# Autodesk Inventor assembly: CanSat
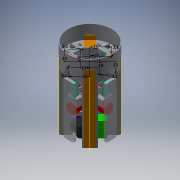
[picture p0: Inventor's stored thumbnail of the model, 180x180]
Saved by Autodesk Inventor 2018.2 (Build 222227000, 227)
## iProperties
Created: 2018-05-01
Part Number: CanSat
Document SubType Name: Assembly
Designer: suchanek
Author: suchanek
## Documents named in this file (25)
- C:\Users\Kuba\Documents\GitHub\CanSatGOSA\CanSat2.0\Schematics\Model\CanSat.iam
- C:\Users\Kuba\Documents\GitHub\CanSatGOSA\CanSat2.0\Schematics\Model\Hull_middle.ipt
- C:\Users\Kuba\Documents\GitHub\CanSatGOSA\CanSat2.0\Schematics\Model\Hull_batt_pillar.ipt
- C:\Users\Kuba\Documents\GitHub\CanSatGOSA\CanSat2.0\Schematics\Model\Circuit.ipt
- C:\Users\Kuba\Documents\GitHub\CanSatGOSA\CanSat2.0\Schematics\Model\Motor_drivers.ipt
- C:\Users\Kuba\Documents\GitHub\CanSatGOSA\CanSat2.0\Schematics\Model\Hull_main.ipt
- C:\Users\Kuba\Documents\GitHub\CanSatGOSA\CanSat2.0\Schematics\Model\Circuit_center.ipt
- C:\Users\Kuba\Documents\GitHub\CanSatGOSA\CanSat2.0\Schematics\Model\Arm.ipt
- C:\Users\Kuba\Documents\GitHub\CanSatGOSA\CanSat2.0\Schematics\Model\Motor_holder.ipt
- C:\Users\Kuba\Documents\GitHub\CanSatGOSA\CanSat2.0\Schematics\Model\Motor.ipt
- C:\Users\Kuba\Documents\GitHub\CanSatGOSA\CanSat2.0\Schematics\Model\Rotor.ipt
- C:\Users\Kuba\Documents\GitHub\CanSatGOSA\CanSat2.0\Schematics\Model\Flight_controler.ipt
- C:\Users\Kuba\Documents\GitHub\CanSatGOSA\CanSat2.0\Schematics\Model\SIM808.ipt
- C:\Users\Kuba\Documents\GitHub\CanSatGOSA\CanSat2.0\Schematics\Model\Batt_pillar.ipt
- C:\Users\Kuba\Documents\GitHub\CanSatGOSA\CanSat2.0\Schematics\Model\Servo.ipt
- C:\Users\Kuba\Documents\GitHub\CanSatGOSA\CanSat2.0\Schematics\Model\Servo_bit.ipt
- C:\Users\Kuba\Documents\GitHub\CanSatGOSA\CanSat2.0\Schematics\Model\Spring.ipt
- C:\Users\Kuba\Documents\GitHub\CanSatGOSA\CanSat2.0\Schematics\Model\Scraper.ipt
- C:\Users\Kuba\Documents\GitHub\CanSatGOSA\CanSat2.0\Schematics\Model\Camera.ipt
- C:\Users\Kuba\Documents\GitHub\CanSatGOSA\CanSat2.0\Schematics\Model\Cam_SD_base.ipt
- C:\Users\Kuba\Documents\GitHub\CanSatGOSA\CanSat2.0\Schematics\Model\Cam_SD_chip.ipt
- C:\Users\Kuba\Documents\GitHub\CanSatGOSA\CanSat2.0\Schematics\Model\Hull_batt_pillar1.ipt
- C:\Users\Kuba\Documents\GitHub\CanSatGOSA\CanSat2.0\Schematics\Model\Hull_batt_pillar3.ipt
- C:\Users\Kuba\Documents\GitHub\CanSatGOSA\CanSat2.0\Schematics\Model\Hull_batt_pillar2.ipt
- C:\Users\Kuba\Documents\GitHub\CanSatGOSA\CanSat2.0\Schematics\Model\Hull_batt_pillar4.ipt
## Components (42 placed, 24 different names)
1. Hull_middle:1 — Rotational:2, Angle:2, Rotational:3, Flush:2, Mate:9
2. Circuit:1 — Rotational:2, Angle:2, Angle:3
3. Motor_drivers:1 — Flush:1, Angle:4, Cylindrical:1, Mate:1
4. Hull_main:1 — Rotational:1, Angle:1, Rotational:3, Angle:3, Flush:1, Angle:4, Cylindrical:1, Rotational:4, Mate:3, Mate:6, Tangent:1, Rotační:8, Rotační:9, Rotační:10, Rotační:11, Rotační:12, Rotační:13, Rotační:14
5. Circuit_center:1 — Flush:2, Mate:9, Tangent:1
6. Flight_controler:1 — Mate:1, Mate:2, Flush:4, Symmetry:1
7. SIM808:1 — Mate:2, Flush:4, Symmetry:1, Mate:7
8. Servo:1 — Rotational:6, Mate:8, Flush:6, Flush:11
9. Servo_bit:1 — Rotational:6, Rigid:3, Angle:11
10. Spring:1 — Rigid:3, Rotational:7
11. Scraper:1 — Rotational:7, Angle:11
12. Camera:1 — Flush:7, Flush:11
13. Cam_SD_base:1 — Flush:8, Angle:12, Flush:10, Angle:13
14. Cam_SD_chip:1 — Flush:10, Angle:13
15. Hull_batt_pillar1:1 — Rotační:8
16. Hull_batt_pillar3:1 — Rotační:9, Rotační:10
17. Hull_batt_pillar2:1 — Rotační:11, Rotační:12
18. Hull_batt_pillar4:1 — Rotační:13, Rotační:14
19. Batt_pillar:1 — Cylindrical:2, Mate:6, Angle:8
20. Hull_batt_pillar:1 — Rotational:1, Angle:1, Cylindrical:2, Angle:8, Angle:10
21. Batt_pillar:2 — Flush:8, Angle:12
22. Hull_batt_pillar:2
23. Batt_pillar:3
24. Hull_batt_pillar:3 — Mate:7
25. Batt_pillar:4
26. Hull_batt_pillar:4 — Angle:9, Mate:8, Flush:6, Flush:7
27. Arm:1 — Rotational:4, Rigid:1
28. Motor_holder:1 — Rigid:1, Rigid:2
29. Motor:1 — Rigid:2, Rotational:5
30. Rotor:1 — Rotational:5
31. Arm:2
32. Motor_holder:2
33. Motor:2
34. Rotor:2
35. Arm:3
36. Motor_holder:3
37. Motor:3
38. Rotor:3
39. Arm:4
40. Motor_holder:4
41. Motor:4
42. Rotor:4
## Component patterns: (4 elements, first: Batt_pillar:1 + Hull_batt_pillar:1), (4 elements, first: Arm:1 + Motor_holder:1 + Motor:1 + Rotor:1)
## Relationships (48: RevoluteJoint 14, Angle 10, Mate 9, Flush 8, WeldJoint 3, CylindricalJoint 2, Symmetry 1, Tangent 1)
- Rotational:1 [RevoluteJoint]: Hull_main:1 ↔ Hull_batt_pillar:1
- Angle:1 (0 deg): Hull_main:1 ↔ Hull_batt_pillar:1
- Rotational:2 [RevoluteJoint]: Hull_middle:1 ↔ Circuit:1
- Angle:2 (0 deg): Hull_middle:1 ↔ Circuit:1
- Rotational:3 [RevoluteJoint]: Hull_middle:1 ↔ Hull_main:1
- Angle:3 (0 deg): Circuit:1 ↔ Hull_main:1
- Flush:1 (12 mm): Motor_drivers:1 ↔ Hull_main:1
- Angle:4 (0 deg): Motor_drivers:1 ↔ Hull_main:1
- Cylindrical:1: Motor_drivers:1 ↔ Hull_main:1
- Flush:2 (3 mm): Hull_middle:1 ↔ Circuit_center:1
- Rotational:4 [RevoluteJoint] (-0.15 mm): Hull_main:1 ↔ Arm:1
- Rigid:1 [WeldJoint]: Arm:1 ↔ Motor_holder:1
- Rigid:2 [WeldJoint]: Motor_holder:1 ↔ Motor:1
- Rotational:5 [RevoluteJoint]: Motor:1 ↔ Rotor:1
- Mate:1 (5 mm): Motor_drivers:1 ↔ Flight_controler:1
- Mate:2 (2 mm): Flight_controler:1 ↔ SIM808:1
- Mate:3: Hull_main:1
- Mate:4
- Mate:5
- Flush:4 (-0.5 mm): Flight_controler:1 ↔ SIM808:1
- Cylindrical:2: Batt_pillar:1 ↔ Hull_batt_pillar:1
- Mate:6: Hull_main:1 ↔ Batt_pillar:1
- Angle:8 (0 deg): Batt_pillar:1 ↔ Hull_batt_pillar:1
- Angle:9 (0 deg): Hull_batt_pillar:4
- Angle:10 (0 deg): Hull_batt_pillar:1
- Symmetry:1: Flight_controler:1 ↔ SIM808:1
- Mate:7: SIM808:1 ↔ Hull_batt_pillar:3
- Rotational:6 [RevoluteJoint]: Servo:1 ↔ Servo_bit:1
- Rigid:3 [WeldJoint]: Servo_bit:1 ↔ Spring:1
- Rotational:7 [RevoluteJoint]: Spring:1 ↔ Scraper:1
- Angle:11 (0 deg): Servo_bit:1 ↔ Scraper:1
- Mate:8: Servo:1 ↔ Hull_batt_pillar:4
- Flush:6: Servo:1 ↔ Hull_batt_pillar:4
- Flush:7: Camera:1 ↔ Hull_batt_pillar:4
- Flush:8: Cam_SD_base:1 ↔ Batt_pillar:2
- Angle:12 (0 deg): Cam_SD_base:1 ↔ Batt_pillar:2
- Flush:10: Cam_SD_base:1 ↔ Cam_SD_chip:1
- Angle:13 (0 deg): Cam_SD_base:1 ↔ Cam_SD_chip:1
- Flush:11: Servo:1 ↔ Camera:1
- Mate:9 (0.245 mm): Hull_middle:1 ↔ Circuit_center:1
- Tangent:1 (-16.4 mm): Hull_main:1 ↔ Circuit_center:1
- Rotační:8 [RevoluteJoint]: Hull_main:1 ↔ Hull_batt_pillar1:1
- Rotační:9 [RevoluteJoint]: Hull_main:1 ↔ Hull_batt_pillar3:1
- Rotační:10 [RevoluteJoint]: Hull_main:1 ↔ Hull_batt_pillar3:1
- Rotační:11 [RevoluteJoint]: Hull_main:1 ↔ Hull_batt_pillar2:1
- Rotační:12 [RevoluteJoint]: Hull_main:1 ↔ Hull_batt_pillar2:1
- Rotační:13 [RevoluteJoint]: Hull_main:1 ↔ Hull_batt_pillar4:1
- Rotační:14 [RevoluteJoint]: Hull_main:1 ↔ Hull_batt_pillar4:1
